# Autodesk Inventor assembly: A2017_T3_04
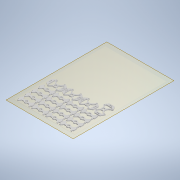
[picture p0: Inventor's stored thumbnail of the model, 180x180]
Saved by Autodesk Inventor 2020 (Build 240168000, 168)
## iProperties
Created: 2021-08-27
Part Number: A2017_T3_04
Document SubType Name: Assembly
Designer: Masato
Author: Masato
## Documents named in this file (4)
- C:\Inventor\SUSTAINA-OP\Cam\A2017_T3_04.iam
- C:\Inventor\SUSTAINA-OP\Cam\DisposableBoard.ipt
- C:\Inventor\SUSTAINA-OP\LowerBody\Ankle\Ankle_front_frame.ipt
- C:\Inventor\SUSTAINA-OP\LowerBody\Leg_joint\Leg_joint_roll_frame.ipt
## Components (21 placed, 3 different names)
1. DisposableBoard:1 — メイト:2, メイト:1, フラッシュ:1, フラッシュ:2, メイト:4, フラッシュ:3, フラッシュ:4, メイト:5, メイト:7
2. Leg_joint_roll_frame:4 — メイト:6, メイト:7, 正接:2
3. Ankle_front_frame:1 — メイト:4, フラッシュ:3, フラッシュ:4, フラッシュ:5
4. Ankle_front_frame:2
5. Ankle_front_frame:3
6. Ankle_front_frame:4
7. Ankle_front_frame:5
8. Ankle_front_frame:6
9. Ankle_front_frame:7
10. Ankle_front_frame:8
11. Ankle_front_frame:9
12. Ankle_front_frame:10
13. Ankle_front_frame:11
14. Ankle_front_frame:12
15. Ankle_front_frame:13 — 正接:1
16. Ankle_front_frame:14
17. Ankle_front_frame:15
18. Ankle_front_frame:16 — メイト:6
19. Leg_joint_roll_frame:1 — メイト:5, フラッシュ:5, 正接:1
20. Leg_joint_roll_frame:2
21. Leg_joint_roll_frame:3 — 正接:2
## Component patterns: (16 elements, first: Ankle_front_frame:1), (3 elements, first: Leg_joint_roll_frame:1)
## Relationships (13: Mate 6, Flush 5, Tangent 2)
- メイト:2 [Mate]: DisposableBoard:1
- メイト:1 [Mate]: DisposableBoard:1
- フラッシュ:1 [Flush]: DisposableBoard:1
- フラッシュ:2 [Flush]: DisposableBoard:1
- メイト:4 [Mate]: DisposableBoard:1 ↔ Ankle_front_frame:1
- フラッシュ:3 [Flush] (2 mm): DisposableBoard:1 ↔ Ankle_front_frame:1
- フラッシュ:4 [Flush] (8 mm): DisposableBoard:1 ↔ Ankle_front_frame:1
- メイト:5 [Mate]: DisposableBoard:1 ↔ Leg_joint_roll_frame:1
- フラッシュ:5 [Flush]: Ankle_front_frame:1 ↔ Leg_joint_roll_frame:1
- 正接:1 [Tangent] (2.5 mm): Ankle_front_frame:13 ↔ Leg_joint_roll_frame:1
- メイト:6 [Mate] (2.5 mm): Leg_joint_roll_frame:4 ↔ Ankle_front_frame:16
- メイト:7 [Mate]: DisposableBoard:1 ↔ Leg_joint_roll_frame:4
- 正接:2 [Tangent] (2.5 mm): Leg_joint_roll_frame:4 ↔ Leg_joint_roll_frame:3
